# Autodesk Inventor assembly: CS_Camera_HD3000
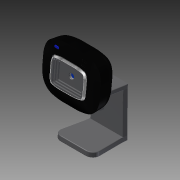
[picture p0: Inventor's stored thumbnail of the model, 180x180]
Saved by Autodesk Inventor 2015 SP1 (Build 190203100, 203)
## iProperties
Category: Control System
Company: Autodesk Inc.
Created: 2014-12-30
Part Number: CS_Camera_HD3000
Document SubType Name: Assembly
Designer: Autodesk Inc.
Catalog Web Link: http://www.microsoft.com/hardware/en-ca/p/lifecam-hd-3000
Vendor: Microsoft Inc.
Author: Autodesk Inc.
## Documents named in this file (3)
- D:\Data Folder\FIRST 2015\KOP_FRC\Control System\CS_Camera_HD3000.iam
- D:\Data Folder\FIRST 2015\KOP_FRC\Control System\CS_Camera_HD3000.ipt
- D:\Data Folder\FIRST 2015\KOP_FRC\Control System\CS_Camera_HD3000_Base_01.ipt
## Components (2 placed, 2 different names)
1. CS_Camera_HD3000:1 — Mate:1, Mate:2
2. CS_Camera_HD3000_Base_01:1 — Mate:1, Mate:2
## Relationships (2: Mate 2)
- Mate:1: CS_Camera_HD3000:1 ↔ CS_Camera_HD3000_Base_01:1
- Mate:2: CS_Camera_HD3000:1 ↔ CS_Camera_HD3000_Base_01:1
